# Autodesk Inventor assembly: Test Stand Assembly
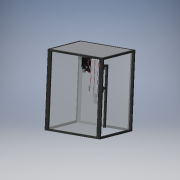
[picture p0: Inventor's stored thumbnail of the model, 180x180]
Saved by Autodesk Inventor 2019 (Build 230136000, 136)
## iProperties
Created: 2021-03-05
Part Number: Test Stand Assembly
Document SubType Name: Assembly
Designer: User
Author: User
## Documents named in this file (12)
- C:\Users\User\Desktop\Test Stand\Test Stand Assembly.iam
- C:\Users\User\Desktop\Test Stand\Base.ipt
- C:\Users\User\Desktop\Test Stand\Perspex shield.ipt
- C:\Users\User\Desktop\Test Stand\Load cell.ipt
- C:\Users\User\Desktop\motor test stand\rocket motor standassembly motor.iam
- C:\Users\User\Desktop\Test Stand\Protoboard.ipt
- C:\Users\User\Desktop\Test Stand\ArduinoUNO .ipt
- C:\Users\User\Desktop\Test Stand\Steel support4.ipt
- C:\Users\User\Desktop\Test Stand\Steel support 5.ipt
- C:\Users\User\Desktop\Test Stand\Steel support 2.ipt
- C:\Users\User\Desktop\Test Stand\support.ipt
- C:\Users\User\Documents\Inventor\Content Center Files\R2019\en-US\CSN EN 28676\ISO 8676 - M8 x 1 x 30CSN EN.ipt
## Components (22 placed, 11 different names)
1. Base:1 — Mate:1, Mate:2, Mate:3, Mate:4, Mate:52, Mate:55, Mate:59, Mate:60
2. Perspex shield:1 — Mate:1, Mate:2, Mate:48, Mate:49, Mate:50, Mate:75, Mate:76
3. Perspex shield:2 — Mate:3, Mate:4, Mate:12, Mate:14, Mate:45, Mate:46, Mate:47, Mate:63
4. rocket motor standassembly motor:1 [sub-assembly] — Mate:74, Mate:77, Mate:78, Rigid:1, Rigid:2, Cylindrical:1, Rigid:3, Rigid:4, Rigid:5, Rigid:6, Cylindrical:2
5. Protoboard:1 — Mate:12, Mate:15, Tangent:2, Mate:57
6. ArduinoUNO :1 — Mate:14, Mate:15, Tangent:2, Mate:58
7. Steel support4:1 — Mate:45, Mate:46, Mate:47, Mate:53, Mate:54, Mate:57, Mate:58
8. Steel support4:2 — Mate:48, Mate:49, Mate:50, Mate:51, Mate:56
9. Steel support 5:1 — Mate:51, Mate:52, Mate:53
10. Steel support 5:2 — Mate:54, Mate:55, Mate:56
11. Steel support 2:1 — Mate:59, Mate:60, Mate:65, Mate:66
12. Load cell:2 — Mate:62, Mate:64, Mate:67, Mate:74
13. Steel support 2:2 — Mate:62, Mate:63, Mate:64, Mate:65, Mate:66, Mate:67
14. support:1 — Mate:75, Mate:76, Mate:77, Mate:78
15. CSN EN 28676 M8 x 1 x 30:1 — Rigid:1
16. CSN EN 28676 M8 x 1 x 30:2 — Cylindrical:1
17. CSN EN 28676 M8 x 1 x 30:3 — Rigid:3
18. CSN EN 28676 M8 x 1 x 30:4 — Cylindrical:2
19. CSN EN 28676 M8 x 1 x 30:5 — Rigid:6
20. CSN EN 28676 M8 x 1 x 30:6 — Rigid:5
21. CSN EN 28676 M8 x 1 x 30:7 — Rigid:4
22. CSN EN 28676 M8 x 1 x 30:8 — Rigid:2
## Relationships (43: Mate 34, WeldJoint 6, CylindricalJoint 2, Tangent 1)
- Mate:1: Base:1 ↔ Perspex shield:1
- Mate:2: Base:1 ↔ Perspex shield:1
- Mate:3: Base:1 ↔ Perspex shield:2
- Mate:4: Base:1 ↔ Perspex shield:2
- Mate:12: Perspex shield:2 ↔ Protoboard:1
- Mate:14: Perspex shield:2 ↔ ArduinoUNO :1
- Mate:15: Protoboard:1 ↔ ArduinoUNO :1
- Tangent:2: Protoboard:1 ↔ ArduinoUNO :1
- Mate:45: Perspex shield:2 ↔ Steel support4:1
- Mate:46: Perspex shield:2 ↔ Steel support4:1
- Mate:47: Perspex shield:2 ↔ Steel support4:1
- Mate:48: Perspex shield:1 ↔ Steel support4:2
- Mate:49: Perspex shield:1 ↔ Steel support4:2
- Mate:50: Perspex shield:1 ↔ Steel support4:2
- Mate:51: Steel support4:2 ↔ Steel support 5:1
- Mate:52: Base:1 ↔ Steel support 5:1
- Mate:53: Steel support4:1 ↔ Steel support 5:1
- Mate:54: Steel support4:1 ↔ Steel support 5:2
- Mate:55: Base:1 ↔ Steel support 5:2
- Mate:56: Steel support4:2 ↔ Steel support 5:2
- Mate:57: Protoboard:1 ↔ Steel support4:1
- Mate:58: ArduinoUNO :1 ↔ Steel support4:1
- Mate:59: Base:1 ↔ Steel support 2:1
- Mate:60: Base:1 ↔ Steel support 2:1
- Mate:62: Load cell:2 ↔ Steel support 2:2
- Mate:63: Perspex shield:2 ↔ Steel support 2:2
- Mate:64: Load cell:2 ↔ Steel support 2:2
- Mate:65: Steel support 2:1 ↔ Steel support 2:2
- Mate:66: Steel support 2:1 ↔ Steel support 2:2
- Mate:67: Load cell:2 ↔ Steel support 2:2
- Mate:74: rocket motor standassembly motor:1 ↔ Load cell:2
- Mate:75: Perspex shield:1 ↔ support:1
- Mate:76: Perspex shield:1 ↔ support:1
- Mate:77: rocket motor standassembly motor:1 ↔ support:1
- Mate:78: rocket motor standassembly motor:1 ↔ support:1
- Rigid:1 [WeldJoint]: rocket motor standassembly motor:1 ↔ CSN EN 28676 M8 x 1 x 30:1
- Rigid:2 [WeldJoint]: rocket motor standassembly motor:1 ↔ CSN EN 28676 M8 x 1 x 30:8
- Cylindrical:1: rocket motor standassembly motor:1 ↔ CSN EN 28676 M8 x 1 x 30:2
- Rigid:3 [WeldJoint]: rocket motor standassembly motor:1 ↔ CSN EN 28676 M8 x 1 x 30:3
- Rigid:4 [WeldJoint]: rocket motor standassembly motor:1 ↔ CSN EN 28676 M8 x 1 x 30:7
- Rigid:5 [WeldJoint]: rocket motor standassembly motor:1 ↔ CSN EN 28676 M8 x 1 x 30:6
- Rigid:6 [WeldJoint]: rocket motor standassembly motor:1 ↔ CSN EN 28676 M8 x 1 x 30:5
- Cylindrical:2: rocket motor standassembly motor:1 ↔ CSN EN 28676 M8 x 1 x 30:4
